# Autodesk Inventor assembly: RPI and PiTFT
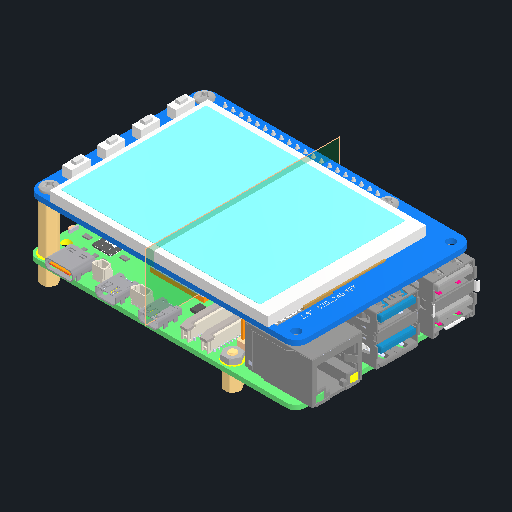
[picture p0: Inventor's stored thumbnail of the model, 512x512]
Saved by Autodesk Inventor 2026 (Build 300175000, 175)
## iProperties
Created: 2025-06-05
Part Number: RPI and PiTFT
Document SubType Name: Assembly
Designer: ckyiu
Author: ckyiu
## Documents named in this file (7)
- C:\Users\ckyiu\Documents\Projects\Chessboard-Design\Assemblies\RPI and PiTFT.iam
- C:\Users\ckyiu\Documents\Projects\Chessboard-Design\Assemblies\Hardware\Raspberry Pi 5.iam
- C:\Users\ckyiu\Documents\Projects\Chessboard-Design\Assemblies\Hardware\PiTFT 2.8in capacitive.ipt
- C:\Users\ckyiu\Documents\Projects\Chessboard-Design\Parts\Standoffs\M2.5 F-M Standoff 6mm.ipt
- C:\Users\ckyiu\Documents\Projects\Chessboard-Design\Parts\Standoffs\M2.5 Nut 1.8mm.ipt
- C:\Users\ckyiu\Documents\Projects\Chessboard-Design\Parts\Standoffs\M2.5 F-F Standoff 16mm.ipt
- C:\Users\ckyiu\Documents\Projects\Chessboard-Design\Parts\Standoffs\M2.5 Screw 6mm.ipt
## Components (13 placed, 6 different names)
1. Raspberry Pi 5:1 [sub-assembly] — Flush:1, Mate:1, Flush:2, Insert:1, Angle:1, Insert:2, Angle:2, Insert:3, Insert:4, Angle:3, Angle:4, Insert:5, Angle:5, Insert:6, Insert:7, Insert:8
2. PiTFT 2.8in capacitive:1 — Flush:1, Mate:1, Flush:2, Insert:9, Insert:10, Insert:11
3. M2.5 F-M Standoff 6mm:1 — Insert:1, Angle:1, Angle:7
4. M2.5 F-M Standoff 6mm:2 — Insert:2, Angle:2, Angle:8
5. M2.5 F-M Standoff 6mm:3 — Insert:4, Angle:3, Angle:6
6. M2.5 F-M Standoff 6mm:4 — Insert:3, Angle:4
7. M2.5 Nut 1.8mm:1 — Insert:5, Angle:5
8. M2.5 F-F Standoff 16mm:1 — Insert:8, Angle:8
9. M2.5 F-F Standoff 16mm:2 — Insert:7, Angle:7
10. M2.5 F-F Standoff 16mm:3 — Insert:6, Angle:6
11. M2.5 Screw 6mm:1 — Insert:9
12. M2.5 Screw 6mm:2 — Insert:10
13. M2.5 Screw 6mm:3 — Insert:11
## Relationships (22: Insert 11, Angle 8, Flush 2, Mate 1)
- Flush:1: Raspberry Pi 5:1 ↔ PiTFT 2.8in capacitive:1
- Mate:1: Raspberry Pi 5:1 ↔ PiTFT 2.8in capacitive:1
- Flush:2: Raspberry Pi 5:1 ↔ PiTFT 2.8in capacitive:1
- Insert:1: Raspberry Pi 5:1 ↔ M2.5 F-M Standoff 6mm:1
- Angle:1 (0 deg): Raspberry Pi 5:1 ↔ M2.5 F-M Standoff 6mm:1
- Insert:2: Raspberry Pi 5:1 ↔ M2.5 F-M Standoff 6mm:2
- Angle:2 (0 deg): Raspberry Pi 5:1 ↔ M2.5 F-M Standoff 6mm:2
- Insert:3: Raspberry Pi 5:1 ↔ M2.5 F-M Standoff 6mm:4
- Insert:4: Raspberry Pi 5:1 ↔ M2.5 F-M Standoff 6mm:3
- Angle:3 (0 deg): Raspberry Pi 5:1 ↔ M2.5 F-M Standoff 6mm:3
- Angle:4 (0 deg): Raspberry Pi 5:1 ↔ M2.5 F-M Standoff 6mm:4
- Insert:5: Raspberry Pi 5:1 ↔ M2.5 Nut 1.8mm:1
- Angle:5 (0 deg): Raspberry Pi 5:1 ↔ M2.5 Nut 1.8mm:1
- Insert:6: Raspberry Pi 5:1 ↔ M2.5 F-F Standoff 16mm:3
- Insert:7: Raspberry Pi 5:1 ↔ M2.5 F-F Standoff 16mm:2
- Insert:8: Raspberry Pi 5:1 ↔ M2.5 F-F Standoff 16mm:1
- Angle:6 (0 deg): M2.5 F-M Standoff 6mm:3 ↔ M2.5 F-F Standoff 16mm:3
- Angle:7 (0 deg): M2.5 F-M Standoff 6mm:1 ↔ M2.5 F-F Standoff 16mm:2
- Angle:8 (0 deg): M2.5 F-M Standoff 6mm:2 ↔ M2.5 F-F Standoff 16mm:1
- Insert:9: PiTFT 2.8in capacitive:1 ↔ M2.5 Screw 6mm:1
- Insert:10: PiTFT 2.8in capacitive:1 ↔ M2.5 Screw 6mm:2
- Insert:11: PiTFT 2.8in capacitive:1 ↔ M2.5 Screw 6mm:3
